# Autodesk Inventor assembly: NeoOnVersa2Stage
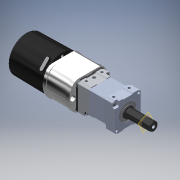
[picture p0: Inventor's stored thumbnail of the model, 180x180]
Saved by Autodesk Inventor 2018 (Build 220112000, 112)
## iProperties
Created: 2016-10-31
Part Number: NeoOnVersa2Stage
Description: STEP AP214
Document SubType Name: Assembly
Designer: user
Mass: 698.532 g
Surface Area: 781.615 cm^2
Volume: 185.532 cm^3
Density: 3.76503 g/cm^3
Sending System: SolidWorks 2016
Preprocessor: SwSTEP 2.0
Title: 217-4973_2stage_BAG.STEP
Revision Number: ANY
## Documents named in this file (15)
- C:\Users\Cooper\Documents\GrabCAD\Infinite Recharge 2020\Build season\180 VERSAPLANETARY\NeoOnVersa2Stage.iam
- C:\Users\Cooper\Documents\GrabCAD\Infinite Recharge 2020\Build season\180 VERSAPLANETARY\217-2625-026 Rev1.ipt
- C:\Users\Cooper\Documents\GrabCAD\Infinite Recharge 2020\Build season\180 VERSAPLANETARY\217-2742-001 Rev4.ipt
- C:\Users\Cooper\Documents\GrabCAD\Infinite Recharge 2020\Build season\180 VERSAPLANETARY\217-2625-003 Rev1.ipt
- C:\Users\Cooper\Documents\GrabCAD\Infinite Recharge 2020\Build season\180 VERSAPLANETARY\832-2250-Base-Kit-Screw_SSA0832-0500ZC.ipt
- C:\Users\Cooper\Documents\GrabCAD\Infinite Recharge 2020\Build season\180 VERSAPLANETARY\217-2625-025 Rev1.ipt
- C:\Users\Cooper\Documents\GrabCAD\Infinite Recharge 2020\Build season\180 VERSAPLANETARY\217-4649-002 Rev1_SSA0832-0500ZC.ipt
- C:\Users\Cooper\Documents\GrabCAD\Infinite Recharge 2020\Build season\180 VERSAPLANETARY\217-4649-006 Rev1_SSA0004-008BA.ipt
- C:\Users\Cooper\Documents\GrabCAD\Infinite Recharge 2020\Build season\180 VERSAPLANETARY\217-2816-001 Rev1.ipt
- C:\Users\Cooper\Documents\GrabCAD\Infinite Recharge 2020\Build season\180 VERSAPLANETARY\217-4649-001 Rev1.ipt
- C:\Users\Cooper\Documents\GrabCAD\Infinite Recharge 2020\Build season\180 VERSAPLANETARY\217-4649-007 Rev1_94105A824.ipt
- C:\Users\Cooper\Documents\GrabCAD\Infinite Recharge 2020\Build season\180 VERSAPLANETARY\217-2625-011 Rev1.ipt
- C:\Users\Cooper\Documents\GrabCAD\Infinite Recharge 2020\Build season\180 VERSAPLANETARY\217-2822-002 Rev4.ipt
- C:\Users\Cooper\Documents\GrabCAD\Infinite Recharge 2020\Build season\180 VERSAPLANETARY\NEO_Adapter_Fixed.ipt
- C:\Users\Cooper\Documents\GrabCAD\Infinite Recharge 2020\Build season\180 VERSAPLANETARY\REV-21-1650.ipt
## Components (18 placed, 17 different names)
1. 217-2625-026 Rev1_1 — Mate:5, Mate:6, Angle:3, Insert:2
2. 217-2742-001 Rev4_3 — Insert:2, Mate:7, Mate:8
3. 217-2625-003 Rev1_5 — Mate:7, Mate:8
4. 832-2250-Base-Kit-Screw_SSA0832-0500ZC_7
5. 832-2250-Base-Kit-Screw_SSA0832-0500ZC_8 — Mate:1
6. 217-2625-025 Rev1_9 — Angle:1
7. 217-4649-002 Rev1_SSA0832-0500ZC_10
8. 217-4649-002 Rev1_SSA0832-0500ZC_11
9. 217-2816-001 Rev1_17 — Mate:3, Mate:4, Angle:2, Mate:5, Mate:6, Angle:3
10. 217-2816-001 Rev1_19 — Mate:3, Mate:4, Angle:2
11. 217-4649-001 Rev1_20
12. 217-4649-007 Rev1_94105A824_21
13. 217-2625-011 Rev1_22
14. 217-4649-006 Rev1_SSA0004-008BA:1
15. 217-4649-006 Rev1_SSA0004-008BA:2
16. 217-2822-002 Rev4:1 — Mate:2
17. NEO_Adapter_Fixed:1 — Mate:1, Angle:1, Mate:2, Insert:1
18. REV-21-1650:1 — Insert:1
## Relationships (13: Mate 8, Angle 3, Insert 2)
- Mate:1: 832-2250-Base-Kit-Screw_SSA0832-0500ZC_8 ↔ NEO_Adapter_Fixed:1
- Angle:1 (0 deg): 217-2625-025 Rev1_9 ↔ NEO_Adapter_Fixed:1
- Mate:2: 217-2822-002 Rev4:1 ↔ NEO_Adapter_Fixed:1
- Insert:1: NEO_Adapter_Fixed:1 ↔ REV-21-1650:1
- Mate:3: 217-2816-001 Rev1_17 ↔ 217-2816-001 Rev1_19
- Mate:4: 217-2816-001 Rev1_17 ↔ 217-2816-001 Rev1_19
- Angle:2 (0 deg): 217-2816-001 Rev1_17 ↔ 217-2816-001 Rev1_19
- Mate:5: 217-2625-026 Rev1_1 ↔ 217-2816-001 Rev1_17
- Mate:6: 217-2625-026 Rev1_1 ↔ 217-2816-001 Rev1_17
- Angle:3 (0 deg): 217-2625-026 Rev1_1 ↔ 217-2816-001 Rev1_17
- Insert:2: 217-2625-026 Rev1_1 ↔ 217-2742-001 Rev4_3
- Mate:7: 217-2742-001 Rev4_3 ↔ 217-2625-003 Rev1_5
- Mate:8: 217-2742-001 Rev4_3 ↔ 217-2625-003 Rev1_5
